# Autodesk Inventor assembly: Top_Slider Assy
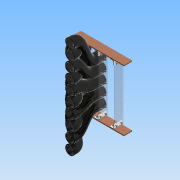
[picture p0: Inventor's stored thumbnail of the model, 180x180]
Saved by Autodesk Inventor 2018.1 (Build 221171000, 171)
## iProperties
Created: 2019-03-18
Part Number: Top_Slider Assy
Document SubType Name: Assembly
Designer: James
Author: James
## Documents named in this file (18)
- C:\Users\admin\Desktop\Ball-Machine\Top Level\Top_Slider Assy.iam
- C:\Users\admin\Desktop\Ball-Machine\Top Level\Top_Slider Piece 1.ipt
- C:\Users\admin\Desktop\Ball-Machine\Top Level\Top_Slider Piece 2.ipt
- C:\Users\admin\Desktop\Ball-Machine\Timing Gate\Timing_Angle Bracket.ipt
- C:\Users\admin\Desktop\Ball-Machine\Timing Gate\Nyloc Nut - M4.ipt
- C:\Users\admin\Desktop\Ball-Machine\Selection Sort\Socket Csk Screw - (A2) - M4 x  12.ipt
- C:\Users\admin\Desktop\Ball-Machine\Top Level\Pipes\Top_Pipe 01.ipt
- C:\Users\admin\Desktop\Ball-Machine\Top Level\Pipes\Top_Pipe 02.ipt
- C:\Users\admin\Desktop\Ball-Machine\Top Level\Pipes\Top_Pipe 03.ipt
- C:\Users\admin\Desktop\Ball-Machine\Top Level\Pipes\Top_Pipe 04.ipt
- C:\Users\admin\Desktop\Ball-Machine\Top Level\Pipes\Top_Pipe 05.ipt
- C:\Users\admin\Desktop\Ball-Machine\Top Level\Pipes\Top_Pipe 06.ipt
- C:\Users\admin\Desktop\Ball-Machine\Top Level\Pipes\Top_Pipe 07.ipt
- C:\Users\admin\Desktop\Ball-Machine\Top Level\Pipes\Top_Pipe 08.ipt
- C:\Users\admin\Desktop\Ball-Machine\Top Level\Pipes\Top_Pipe 09.ipt
- C:\Users\admin\Desktop\Ball-Machine\Top Level\Pipes\Top_Pipe 10.ipt
- C:\Users\admin\Desktop\Ball-Machine\Selection Sort\Socket Csk Screw - (A2) - M4 x  16.ipt
- C:\Users\admin\Desktop\Ball-Machine\Selection Sort\Socket Cap Screw - Standard - (A2) - M4 x 16.ipt
## Components (109 placed, 17 different names)
1. Top_Slider Piece 1:1 — Mate:1, Mate:2, Flush:6, Flush:7, Mate:25, Mate:75, Mate:76, Tangent:18, Angle:6, Mate:77, Mate:78, Tangent:19, Angle:7, Mate:79, Mate:80, Tangent:20, Angle:8, Mate:81, Mate:82, Tangent:21, Angle:9, Mate:83, Mate:84, Tangent:22, Angle:10, Mate:85, Mate:86, Flush:26, Mate:89, Mate:90, Mate:123, Mate:134
2. Top_Slider Piece 2:1 — Flush:1, Flush:2, Flush:3, Mate:1, Flush:4, Flush:5, Flush:6, Mate:3, Mate:4, Mate:11, Mate:12, Mate:13, Mate:14, Mate:15, Mate:16, Mate:17, Mate:18, Mate:19, Mate:60, Mate:61, Mate:62, Mate:63, Mate:64, Tangent:2, Tangent:3, Tangent:4, Tangent:5, Tangent:10, Tangent:12
3. Top_Slider Piece 1:2 — Flush:7, Flush:8, Mate:3, Mate:24, Mate:65, Mate:66, Tangent:13, Mate:67, Mate:68, Mate:69, Mate:70, Mate:71, Mate:72, Mate:73, Mate:74, Tangent:14, Tangent:15, Tangent:16, Tangent:17, Angle:2, Angle:3, Angle:4, Angle:5, Mate:87, Mate:88, Flush:24, Mate:91, Mate:92, Mate:124, Mate:125, Mate:129, Mate:132, Mate:135, Mate:138
4. Top_Slider Piece 1:3 — Flush:8, Mate:4, Mate:23, Mate:126, Mate:127, Mate:128, Mate:133, Mate:136, Mate:137
5. Top_Slider Piece 2:2 — Mate:2, Flush:4, Flush:5, Mate:5, Mate:6, Mate:7, Flush:9, Flush:10, Mate:8, Mate:9, Mate:10, Mate:20, Mate:21, Mate:22, Mate:27, Tangent:1, Tangent:6, Tangent:7, Tangent:8, Tangent:9, Tangent:11
6. Nyloc Nut - M4:34 — Mate:97, Mate:98
7. Socket Cap Screw - Standard - (A2) - M4 x 16:1 — Mate:97, Mate:98, Flush:27, Mate:121, Mate:123
8. Nyloc Nut - M4:35
9. Socket Cap Screw - Standard - (A2) - M4 x 16:2 — Flush:27, Mate:122
10. Nyloc Nut - M4:36
11. Socket Cap Screw - Standard - (A2) - M4 x 16:3 — Flush:28, Mate:124, Mate:138
12. Nyloc Nut - M4:37
13. Socket Cap Screw - Standard - (A2) - M4 x 16:4 — Flush:28, Mate:125
14. Nyloc Nut - M4:38
15. Socket Cap Screw - Standard - (A2) - M4 x 16:5 — Flush:29, Mate:126, Mate:137
16. Nyloc Nut - M4:39
17. Socket Cap Screw - Standard - (A2) - M4 x 16:6 — Flush:29, Mate:127
18. Nyloc Nut - M4:40
19. Socket Cap Screw - Standard - (A2) - M4 x 16:7 — Flush:30, Mate:129, Mate:135
20. Nyloc Nut - M4:41
21. Socket Cap Screw - Standard - (A2) - M4 x 16:8 — Flush:30, Mate:132
22. Nyloc Nut - M4:42
23. Socket Cap Screw - Standard - (A2) - M4 x 16:9 — Flush:31, Mate:130, Mate:134
24. Nyloc Nut - M4:43
25. Socket Cap Screw - Standard - (A2) - M4 x 16:10 — Flush:31, Mate:131
26. Nyloc Nut - M4:44
27. Socket Cap Screw - Standard - (A2) - M4 x 16:11 — Flush:32, Mate:128, Mate:136
28. Nyloc Nut - M4:45
29. Socket Cap Screw - Standard - (A2) - M4 x 16:12 — Flush:32, Mate:133
30. Timing_Angle Bracket:1 — Mate:5, Mate:6, Mate:7, Flush:9, Flush:10, Mate:25, Mate:29, Mate:54, Mate:121, Mate:122
31. Timing_Angle Bracket:2 — Mate:8, Mate:9, Mate:10, Mate:24, Mate:55, Mate:56
32. Timing_Angle Bracket:3 — Mate:11, Mate:12, Mate:13, Mate:59, Mate:130, Mate:131
33. Timing_Angle Bracket:4 — Mate:14, Mate:15, Mate:16
34. Timing_Angle Bracket:5 — Mate:20, Mate:21, Mate:22, Mate:23, Mate:57, Mate:58
35. Timing_Angle Bracket:6 — Mate:17, Mate:18, Mate:19
36. Nyloc Nut - M4:1 — Mate:28, Mate:29
37. Socket Csk Screw - (A2) - M4 x  12:1 — Mate:27, Tangent:1, Mate:28
38. Nyloc Nut - M4:2 — Flush:11, Mate:31
39. Socket Csk Screw - (A2) - M4 x  12:2 — Flush:11, Mate:31, Mate:54, Tangent:6
40. Nyloc Nut - M4:3
41. Socket Csk Screw - (A2) - M4 x  12:3 — Mate:55, Tangent:7
42. Nyloc Nut - M4:4
43. Socket Csk Screw - (A2) - M4 x  12:4 — Mate:56, Tangent:8
44. Nyloc Nut - M4:5
45. Socket Csk Screw - (A2) - M4 x  12:5 — Mate:57, Tangent:11
46. Nyloc Nut - M4:6
47. Socket Csk Screw - (A2) - M4 x  12:6 — Mate:64, Tangent:12
48. Nyloc Nut - M4:8
49. Socket Csk Screw - (A2) - M4 x  12:8 — Mate:58, Tangent:9
50. Nyloc Nut - M4:9
51. Socket Csk Screw - (A2) - M4 x  12:9 — Mate:63, Tangent:10
52. Nyloc Nut - M4:10
53. Socket Csk Screw - (A2) - M4 x  12:10 — Mate:61, Tangent:2
54. Nyloc Nut - M4:11
55. Socket Csk Screw - (A2) - M4 x  12:11 — Mate:62, Tangent:3
56. Nyloc Nut - M4:12
57. Socket Csk Screw - (A2) - M4 x  12:12 — Mate:60, Tangent:5
58. Nyloc Nut - M4:13
59. Socket Csk Screw - (A2) - M4 x  12:13 — Mate:59, Tangent:4
60. Top_Pipe 01:1 — Mate:65, Mate:66, Tangent:13, Angle:1
61. Top_Pipe 02:1 — Mate:67, Mate:68, Tangent:17, Angle:2
62. Top_Pipe 03:1 — Mate:69, Mate:70, Tangent:16, Angle:3
63. Top_Pipe 04:1 — Mate:71, Mate:72, Tangent:15, Angle:4
64. Top_Pipe 05:1 — Mate:73, Mate:74, Tangent:14, Angle:5
65. Top_Pipe 06:1 — Mate:75, Mate:76, Tangent:18, Angle:6
66. Top_Pipe 07:1 — Mate:77, Mate:78, Tangent:19, Angle:7
67. Top_Pipe 08:1 — Mate:79, Mate:80, Tangent:20, Angle:8
68. Top_Pipe 09:1 — Mate:81, Mate:82, Tangent:21, Angle:9
69. Top_Pipe 10:1 — Mate:83, Mate:84, Tangent:22, Angle:10
70. Socket Csk Screw - (A2) - M4 x  16:3 — Mate:87, Flush:23, Flush:24, Mate:93
71. Socket Csk Screw - (A2) - M4 x  16:4 — Mate:88, Flush:23, Mate:94
72. Nyloc Nut - M4:15 — Mate:89, Mate:95
73. Socket Csk Screw - (A2) - M4 x  16:1 — Mate:85, Flush:25, Flush:26, Mate:95
74. Nyloc Nut - M4:14 — Mate:90, Mate:96
75. Socket Csk Screw - (A2) - M4 x  16:2 — Mate:86, Flush:25, Mate:96
76. Nyloc Nut - M4:17 — Mate:92, Mate:94
77. Nyloc Nut - M4:16 — Mate:91, Mate:93
78. Socket Csk Screw - (A2) - M4 x  16:5
79. Socket Csk Screw - (A2) - M4 x  16:6
80. Nyloc Nut - M4:18
81. Socket Csk Screw - (A2) - M4 x  16:7
82. Nyloc Nut - M4:19
83. Socket Csk Screw - (A2) - M4 x  16:8
84. Nyloc Nut - M4:20
85. Nyloc Nut - M4:21
86. Socket Csk Screw - (A2) - M4 x  16:9
87. Socket Csk Screw - (A2) - M4 x  16:10
88. Nyloc Nut - M4:22
89. Socket Csk Screw - (A2) - M4 x  16:11
90. Nyloc Nut - M4:23
91. Socket Csk Screw - (A2) - M4 x  16:12
92. Nyloc Nut - M4:24
93. Nyloc Nut - M4:25
94. Socket Csk Screw - (A2) - M4 x  16:13
95. Socket Csk Screw - (A2) - M4 x  16:14
96. Nyloc Nut - M4:26
97. Socket Csk Screw - (A2) - M4 x  16:15
98. Nyloc Nut - M4:27
99. Socket Csk Screw - (A2) - M4 x  16:16
100. Nyloc Nut - M4:28
101. Nyloc Nut - M4:29
102. Socket Csk Screw - (A2) - M4 x  16:17
103. Socket Csk Screw - (A2) - M4 x  16:18
104. Nyloc Nut - M4:30
105. Socket Csk Screw - (A2) - M4 x  16:19
106. Nyloc Nut - M4:31
107. Socket Csk Screw - (A2) - M4 x  16:20
108. Nyloc Nut - M4:32
109. Nyloc Nut - M4:33
## Component patterns: (5 elements, first: Socket Csk Screw - (A2) - M4 x  16:3 + Socket Csk Screw - (A2) - M4 x  16:4 + Nyloc Nut - M4:15 + Socket Csk Screw - (A2) - M4 x  16:1 + Nyloc Nut - M4:14 + Socket Csk Screw - (A2) - M4 x  16:2 + Nyloc Nut - M4:17 + Nyloc Nut - M4:16)
## Relationships (198: Mate 135, Flush 31, Tangent 22, Angle 10)
- Flush:1: Top_Slider Piece 2:1
- Flush:2: Top_Slider Piece 2:1
- Flush:3: Top_Slider Piece 2:1
- Mate:1: Top_Slider Piece 1:1 ↔ Top_Slider Piece 2:1
- Mate:2: Top_Slider Piece 1:1 ↔ Top_Slider Piece 2:2
- Flush:4: Top_Slider Piece 2:1 ↔ Top_Slider Piece 2:2
- Flush:5: Top_Slider Piece 2:1 ↔ Top_Slider Piece 2:2
- Flush:6: Top_Slider Piece 1:1 ↔ Top_Slider Piece 2:1
- Flush:7: Top_Slider Piece 1:1 ↔ Top_Slider Piece 1:2
- Flush:8: Top_Slider Piece 1:2 ↔ Top_Slider Piece 1:3
- Mate:3: Top_Slider Piece 2:1 ↔ Top_Slider Piece 1:2
- Mate:4: Top_Slider Piece 2:1 ↔ Top_Slider Piece 1:3
- Mate:5: Top_Slider Piece 2:2 ↔ Timing_Angle Bracket:1
- Mate:6: Top_Slider Piece 2:2 ↔ Timing_Angle Bracket:1
- Mate:7: Top_Slider Piece 2:2 ↔ Timing_Angle Bracket:1
- Flush:9: Top_Slider Piece 2:2 ↔ Timing_Angle Bracket:1
- Flush:10: Top_Slider Piece 2:2 ↔ Timing_Angle Bracket:1
- Mate:8: Top_Slider Piece 2:2 ↔ Timing_Angle Bracket:2
- Mate:9: Top_Slider Piece 2:2 ↔ Timing_Angle Bracket:2
- Mate:10: Top_Slider Piece 2:2 ↔ Timing_Angle Bracket:2
- Mate:11: Top_Slider Piece 2:1 ↔ Timing_Angle Bracket:3
- Mate:12: Top_Slider Piece 2:1 ↔ Timing_Angle Bracket:3
- Mate:13: Top_Slider Piece 2:1 ↔ Timing_Angle Bracket:3
- Mate:14: Top_Slider Piece 2:1 ↔ Timing_Angle Bracket:4
- Mate:15: Top_Slider Piece 2:1 ↔ Timing_Angle Bracket:4
- Mate:16: Top_Slider Piece 2:1 ↔ Timing_Angle Bracket:4
- Mate:17: Top_Slider Piece 2:1 ↔ Timing_Angle Bracket:6
- Mate:18: Top_Slider Piece 2:1 ↔ Timing_Angle Bracket:6
- Mate:19: Top_Slider Piece 2:1 ↔ Timing_Angle Bracket:6
- Mate:20: Top_Slider Piece 2:2 ↔ Timing_Angle Bracket:5
- Mate:21: Top_Slider Piece 2:2 ↔ Timing_Angle Bracket:5
- Mate:22: Top_Slider Piece 2:2 ↔ Timing_Angle Bracket:5
- Mate:23: Top_Slider Piece 1:3 ↔ Timing_Angle Bracket:5
- Mate:24: Top_Slider Piece 1:2 ↔ Timing_Angle Bracket:2
- Mate:25: Top_Slider Piece 1:1 ↔ Timing_Angle Bracket:1
- Mate:27: Top_Slider Piece 2:2 ↔ Socket Csk Screw - (A2) - M4 x  12:1
- Tangent:1: Top_Slider Piece 2:2 ↔ Socket Csk Screw - (A2) - M4 x  12:1
- Mate:28: Nyloc Nut - M4:1 ↔ Socket Csk Screw - (A2) - M4 x  12:1
- Mate:29: Timing_Angle Bracket:1 ↔ Nyloc Nut - M4:1
- [Mate]: Nyloc Nut - M4:2 ↔ Socket Csk Screw - (A2) - M4 x  12:2
- Flush:11 (7.78 mm): Nyloc Nut - M4:2 ↔ Socket Csk Screw - (A2) - M4 x  12:2
- Mate:31: Nyloc Nut - M4:2 ↔ Socket Csk Screw - (A2) - M4 x  12:2
- [Mate]: Nyloc Nut - M4:3 ↔ Socket Csk Screw - (A2) - M4 x  12:3
- [Flush] (7.78 mm): Nyloc Nut - M4:3 ↔ Socket Csk Screw - (A2) - M4 x  12:3
- [Mate]: Nyloc Nut - M4:3 ↔ Socket Csk Screw - (A2) - M4 x  12:3
- [Mate]: Nyloc Nut - M4:4 ↔ Socket Csk Screw - (A2) - M4 x  12:4
- [Flush] (7.78 mm): Nyloc Nut - M4:4 ↔ Socket Csk Screw - (A2) - M4 x  12:4
- [Mate]: Nyloc Nut - M4:4 ↔ Socket Csk Screw - (A2) - M4 x  12:4
- [Mate]: Nyloc Nut - M4:5 ↔ Socket Csk Screw - (A2) - M4 x  12:5
- [Flush] (7.78 mm): Nyloc Nut - M4:5 ↔ Socket Csk Screw - (A2) - M4 x  12:5
- [Mate]: Nyloc Nut - M4:5 ↔ Socket Csk Screw - (A2) - M4 x  12:5
- [Mate]: Nyloc Nut - M4:6 ↔ Socket Csk Screw - (A2) - M4 x  12:6
- [Flush] (7.78 mm): Nyloc Nut - M4:6 ↔ Socket Csk Screw - (A2) - M4 x  12:6
- [Mate]: Nyloc Nut - M4:6 ↔ Socket Csk Screw - (A2) - M4 x  12:6
- [Mate]: Nyloc Nut - M4:8 ↔ Socket Csk Screw - (A2) - M4 x  12:8
- [Flush] (7.78 mm): Nyloc Nut - M4:8 ↔ Socket Csk Screw - (A2) - M4 x  12:8
- [Mate]: Nyloc Nut - M4:8 ↔ Socket Csk Screw - (A2) - M4 x  12:8
- [Mate]: Nyloc Nut - M4:9 ↔ Socket Csk Screw - (A2) - M4 x  12:9
- [Flush] (7.78 mm): Nyloc Nut - M4:9 ↔ Socket Csk Screw - (A2) - M4 x  12:9
- [Mate]: Nyloc Nut - M4:9 ↔ Socket Csk Screw - (A2) - M4 x  12:9
- [Mate]: Nyloc Nut - M4:10 ↔ Socket Csk Screw - (A2) - M4 x  12:10
- [Flush] (7.78 mm): Nyloc Nut - M4:10 ↔ Socket Csk Screw - (A2) - M4 x  12:10
- [Mate]: Nyloc Nut - M4:10 ↔ Socket Csk Screw - (A2) - M4 x  12:10
- [Mate]: Nyloc Nut - M4:11 ↔ Socket Csk Screw - (A2) - M4 x  12:11
- [Flush] (7.78 mm): Nyloc Nut - M4:11 ↔ Socket Csk Screw - (A2) - M4 x  12:11
- [Mate]: Nyloc Nut - M4:11 ↔ Socket Csk Screw - (A2) - M4 x  12:11
- [Mate]: Nyloc Nut - M4:12 ↔ Socket Csk Screw - (A2) - M4 x  12:12
- [Flush] (7.78 mm): Nyloc Nut - M4:12 ↔ Socket Csk Screw - (A2) - M4 x  12:12
- [Mate]: Nyloc Nut - M4:12 ↔ Socket Csk Screw - (A2) - M4 x  12:12
- [Mate]: Nyloc Nut - M4:13 ↔ Socket Csk Screw - (A2) - M4 x  12:13
- [Flush] (7.78 mm): Nyloc Nut - M4:13 ↔ Socket Csk Screw - (A2) - M4 x  12:13
- [Mate]: Nyloc Nut - M4:13 ↔ Socket Csk Screw - (A2) - M4 x  12:13
- Mate:54: Timing_Angle Bracket:1 ↔ Socket Csk Screw - (A2) - M4 x  12:2
- Mate:55: Timing_Angle Bracket:2 ↔ Socket Csk Screw - (A2) - M4 x  12:3
- Mate:56: Timing_Angle Bracket:2 ↔ Socket Csk Screw - (A2) - M4 x  12:4
- Mate:57: Timing_Angle Bracket:5 ↔ Socket Csk Screw - (A2) - M4 x  12:5
- Mate:58: Timing_Angle Bracket:5 ↔ Socket Csk Screw - (A2) - M4 x  12:8
- Mate:59: Timing_Angle Bracket:3 ↔ Socket Csk Screw - (A2) - M4 x  12:13
- Mate:60: Top_Slider Piece 2:1 ↔ Socket Csk Screw - (A2) - M4 x  12:12
- Mate:61: Top_Slider Piece 2:1 ↔ Socket Csk Screw - (A2) - M4 x  12:10
- Mate:62: Top_Slider Piece 2:1 ↔ Socket Csk Screw - (A2) - M4 x  12:11
- Mate:63: Top_Slider Piece 2:1 ↔ Socket Csk Screw - (A2) - M4 x  12:9
- Mate:64: Top_Slider Piece 2:1 ↔ Socket Csk Screw - (A2) - M4 x  12:6
- Tangent:2: Top_Slider Piece 2:1 ↔ Socket Csk Screw - (A2) - M4 x  12:10
- Tangent:3: Top_Slider Piece 2:1 ↔ Socket Csk Screw - (A2) - M4 x  12:11
- Tangent:4: Top_Slider Piece 2:1 ↔ Socket Csk Screw - (A2) - M4 x  12:13
- Tangent:5: Top_Slider Piece 2:1 ↔ Socket Csk Screw - (A2) - M4 x  12:12
- Tangent:6: Top_Slider Piece 2:2 ↔ Socket Csk Screw - (A2) - M4 x  12:2
- Tangent:7: Top_Slider Piece 2:2 ↔ Socket Csk Screw - (A2) - M4 x  12:3
- Tangent:8: Top_Slider Piece 2:2 ↔ Socket Csk Screw - (A2) - M4 x  12:4
- Tangent:9: Top_Slider Piece 2:2 ↔ Socket Csk Screw - (A2) - M4 x  12:8
- Tangent:10: Top_Slider Piece 2:1 ↔ Socket Csk Screw - (A2) - M4 x  12:9
- Tangent:11: Top_Slider Piece 2:2 ↔ Socket Csk Screw - (A2) - M4 x  12:5
- Tangent:12: Top_Slider Piece 2:1 ↔ Socket Csk Screw - (A2) - M4 x  12:6
- Mate:65: Top_Slider Piece 1:2 ↔ Top_Pipe 01:1
- Mate:66: Top_Slider Piece 1:2 ↔ Top_Pipe 01:1
- Tangent:13: Top_Slider Piece 1:2 ↔ Top_Pipe 01:1
- Angle:1 (180 deg): Top_Pipe 01:1
- Mate:67: Top_Slider Piece 1:2 ↔ Top_Pipe 02:1
- Mate:68: Top_Slider Piece 1:2 ↔ Top_Pipe 02:1
- Mate:69: Top_Slider Piece 1:2 ↔ Top_Pipe 03:1
- Mate:70: Top_Slider Piece 1:2 ↔ Top_Pipe 03:1
- Mate:71: Top_Slider Piece 1:2 ↔ Top_Pipe 04:1
- Mate:72: Top_Slider Piece 1:2 ↔ Top_Pipe 04:1
- Mate:73: Top_Slider Piece 1:2 ↔ Top_Pipe 05:1
- Mate:74: Top_Slider Piece 1:2 ↔ Top_Pipe 05:1
- Tangent:14: Top_Slider Piece 1:2 ↔ Top_Pipe 05:1
- Tangent:15: Top_Slider Piece 1:2 ↔ Top_Pipe 04:1
- Tangent:16: Top_Slider Piece 1:2 ↔ Top_Pipe 03:1
- Tangent:17: Top_Slider Piece 1:2 ↔ Top_Pipe 02:1
- Angle:2 (0 deg): Top_Slider Piece 1:2 ↔ Top_Pipe 02:1
- Angle:3 (0 deg): Top_Slider Piece 1:2 ↔ Top_Pipe 03:1
- Angle:4 (0 deg): Top_Slider Piece 1:2 ↔ Top_Pipe 04:1
- Angle:5 (0 deg): Top_Slider Piece 1:2 ↔ Top_Pipe 05:1
- Mate:75: Top_Slider Piece 1:1 ↔ Top_Pipe 06:1
- Mate:76: Top_Slider Piece 1:1 ↔ Top_Pipe 06:1
- Tangent:18: Top_Slider Piece 1:1 ↔ Top_Pipe 06:1
- Angle:6 (180 deg): Top_Slider Piece 1:1 ↔ Top_Pipe 06:1
- Mate:77: Top_Slider Piece 1:1 ↔ Top_Pipe 07:1
- Mate:78: Top_Slider Piece 1:1 ↔ Top_Pipe 07:1
- Tangent:19: Top_Slider Piece 1:1 ↔ Top_Pipe 07:1
- Angle:7 (0 deg): Top_Slider Piece 1:1 ↔ Top_Pipe 07:1
- Mate:79: Top_Slider Piece 1:1 ↔ Top_Pipe 08:1
- Mate:80: Top_Slider Piece 1:1 ↔ Top_Pipe 08:1
- Tangent:20: Top_Slider Piece 1:1 ↔ Top_Pipe 08:1
- Angle:8 (0 deg): Top_Slider Piece 1:1 ↔ Top_Pipe 08:1
- Mate:81: Top_Slider Piece 1:1 ↔ Top_Pipe 09:1
- Mate:82: Top_Slider Piece 1:1 ↔ Top_Pipe 09:1
- Tangent:21: Top_Slider Piece 1:1 ↔ Top_Pipe 09:1
- Angle:9 (0 deg): Top_Slider Piece 1:1 ↔ Top_Pipe 09:1
- Mate:83: Top_Slider Piece 1:1 ↔ Top_Pipe 10:1
- Mate:84: Top_Slider Piece 1:1 ↔ Top_Pipe 10:1
- Tangent:22: Top_Slider Piece 1:1 ↔ Top_Pipe 10:1
- Angle:10 (0 deg): Top_Slider Piece 1:1 ↔ Top_Pipe 10:1
- Mate:85: Top_Slider Piece 1:1 ↔ Socket Csk Screw - (A2) - M4 x  16:1
- Mate:86: Top_Slider Piece 1:1 ↔ Socket Csk Screw - (A2) - M4 x  16:2
- Mate:87: Top_Slider Piece 1:2 ↔ Socket Csk Screw - (A2) - M4 x  16:3
- Mate:88: Top_Slider Piece 1:2 ↔ Socket Csk Screw - (A2) - M4 x  16:4
- Flush:23: Socket Csk Screw - (A2) - M4 x  16:3 ↔ Socket Csk Screw - (A2) - M4 x  16:4
- Flush:24 (-5 mm): Top_Slider Piece 1:2 ↔ Socket Csk Screw - (A2) - M4 x  16:3
- Flush:25: Socket Csk Screw - (A2) - M4 x  16:1 ↔ Socket Csk Screw - (A2) - M4 x  16:2
- Flush:26 (-5 mm): Top_Slider Piece 1:1 ↔ Socket Csk Screw - (A2) - M4 x  16:1
- Mate:89: Top_Slider Piece 1:1 ↔ Nyloc Nut - M4:15
- Mate:90: Top_Slider Piece 1:1 ↔ Nyloc Nut - M4:14
- Mate:91: Top_Slider Piece 1:2 ↔ Nyloc Nut - M4:16
- Mate:92: Top_Slider Piece 1:2 ↔ Nyloc Nut - M4:17
- Mate:93: Socket Csk Screw - (A2) - M4 x  16:3 ↔ Nyloc Nut - M4:16
- Mate:94: Socket Csk Screw - (A2) - M4 x  16:4 ↔ Nyloc Nut - M4:17
- Mate:95: Nyloc Nut - M4:15 ↔ Socket Csk Screw - (A2) - M4 x  16:1
- Mate:96: Nyloc Nut - M4:14 ↔ Socket Csk Screw - (A2) - M4 x  16:2
- Mate:97: Nyloc Nut - M4:34 ↔ Socket Cap Screw - Standard - (A2) - M4 x 16:1
- Mate:98 (8 mm): Nyloc Nut - M4:34 ↔ Socket Cap Screw - Standard - (A2) - M4 x 16:1
- [Mate]: Nyloc Nut - M4:35 ↔ Socket Cap Screw - Standard - (A2) - M4 x 16:2
- [Mate] (8 mm): Nyloc Nut - M4:35 ↔ Socket Cap Screw - Standard - (A2) - M4 x 16:2
- [Mate]: Nyloc Nut - M4:36 ↔ Socket Cap Screw - Standard - (A2) - M4 x 16:3
- [Mate] (8 mm): Nyloc Nut - M4:36 ↔ Socket Cap Screw - Standard - (A2) - M4 x 16:3
- [Mate]: Nyloc Nut - M4:37 ↔ Socket Cap Screw - Standard - (A2) - M4 x 16:4
- [Mate] (8 mm): Nyloc Nut - M4:37 ↔ Socket Cap Screw - Standard - (A2) - M4 x 16:4
- [Mate]: Nyloc Nut - M4:38 ↔ Socket Cap Screw - Standard - (A2) - M4 x 16:5
- [Mate] (8 mm): Nyloc Nut - M4:38 ↔ Socket Cap Screw - Standard - (A2) - M4 x 16:5
- [Mate]: Nyloc Nut - M4:39 ↔ Socket Cap Screw - Standard - (A2) - M4 x 16:6
- [Mate] (8 mm): Nyloc Nut - M4:39 ↔ Socket Cap Screw - Standard - (A2) - M4 x 16:6
- [Mate]: Nyloc Nut - M4:40 ↔ Socket Cap Screw - Standard - (A2) - M4 x 16:7
- [Mate] (8 mm): Nyloc Nut - M4:40 ↔ Socket Cap Screw - Standard - (A2) - M4 x 16:7
- [Mate]: Nyloc Nut - M4:41 ↔ Socket Cap Screw - Standard - (A2) - M4 x 16:8
- [Mate] (8 mm): Nyloc Nut - M4:41 ↔ Socket Cap Screw - Standard - (A2) - M4 x 16:8
- [Mate]: Nyloc Nut - M4:42 ↔ Socket Cap Screw - Standard - (A2) - M4 x 16:9
- [Mate] (8 mm): Nyloc Nut - M4:42 ↔ Socket Cap Screw - Standard - (A2) - M4 x 16:9
- [Mate]: Nyloc Nut - M4:43 ↔ Socket Cap Screw - Standard - (A2) - M4 x 16:10
- [Mate] (8 mm): Nyloc Nut - M4:43 ↔ Socket Cap Screw - Standard - (A2) - M4 x 16:10
- [Mate]: Nyloc Nut - M4:44 ↔ Socket Cap Screw - Standard - (A2) - M4 x 16:11
- [Mate] (8 mm): Nyloc Nut - M4:44 ↔ Socket Cap Screw - Standard - (A2) - M4 x 16:11
- [Mate]: Nyloc Nut - M4:45 ↔ Socket Cap Screw - Standard - (A2) - M4 x 16:12
- [Mate] (8 mm): Nyloc Nut - M4:45 ↔ Socket Cap Screw - Standard - (A2) - M4 x 16:12
- Flush:27: Socket Cap Screw - Standard - (A2) - M4 x 16:1 ↔ Socket Cap Screw - Standard - (A2) - M4 x 16:2
- Mate:121: Socket Cap Screw - Standard - (A2) - M4 x 16:1 ↔ Timing_Angle Bracket:1
- Mate:122: Socket Cap Screw - Standard - (A2) - M4 x 16:2 ↔ Timing_Angle Bracket:1
- Mate:123: Top_Slider Piece 1:1 ↔ Socket Cap Screw - Standard - (A2) - M4 x 16:1
- Flush:28: Socket Cap Screw - Standard - (A2) - M4 x 16:3 ↔ Socket Cap Screw - Standard - (A2) - M4 x 16:4
- Flush:29: Socket Cap Screw - Standard - (A2) - M4 x 16:5 ↔ Socket Cap Screw - Standard - (A2) - M4 x 16:6
- Mate:124: Top_Slider Piece 1:2 ↔ Socket Cap Screw - Standard - (A2) - M4 x 16:3
- Mate:125: Top_Slider Piece 1:2 ↔ Socket Cap Screw - Standard - (A2) - M4 x 16:4
- Mate:126: Top_Slider Piece 1:3 ↔ Socket Cap Screw - Standard - (A2) - M4 x 16:5
- Mate:127: Top_Slider Piece 1:3 ↔ Socket Cap Screw - Standard - (A2) - M4 x 16:6
- Flush:30: Socket Cap Screw - Standard - (A2) - M4 x 16:7 ↔ Socket Cap Screw - Standard - (A2) - M4 x 16:8
- Flush:31: Socket Cap Screw - Standard - (A2) - M4 x 16:9 ↔ Socket Cap Screw - Standard - (A2) - M4 x 16:10
- Flush:32: Socket Cap Screw - Standard - (A2) - M4 x 16:11 ↔ Socket Cap Screw - Standard - (A2) - M4 x 16:12
- Mate:128: Top_Slider Piece 1:3 ↔ Socket Cap Screw - Standard - (A2) - M4 x 16:11
- Mate:129: Top_Slider Piece 1:2 ↔ Socket Cap Screw - Standard - (A2) - M4 x 16:7
- Mate:130: Socket Cap Screw - Standard - (A2) - M4 x 16:9 ↔ Timing_Angle Bracket:3
- Mate:131: Socket Cap Screw - Standard - (A2) - M4 x 16:10 ↔ Timing_Angle Bracket:3
- Mate:132: Top_Slider Piece 1:2 ↔ Socket Cap Screw - Standard - (A2) - M4 x 16:8
- Mate:133: Top_Slider Piece 1:3 ↔ Socket Cap Screw - Standard - (A2) - M4 x 16:12
- Mate:134: Top_Slider Piece 1:1 ↔ Socket Cap Screw - Standard - (A2) - M4 x 16:9
- Mate:135: Top_Slider Piece 1:2 ↔ Socket Cap Screw - Standard - (A2) - M4 x 16:7
- Mate:136: Top_Slider Piece 1:3 ↔ Socket Cap Screw - Standard - (A2) - M4 x 16:11
- Mate:137: Top_Slider Piece 1:3 ↔ Socket Cap Screw - Standard - (A2) - M4 x 16:5
- Mate:138: Top_Slider Piece 1:2 ↔ Socket Cap Screw - Standard - (A2) - M4 x 16:3
## Named parameters: d41_d39 = 0 mm, d44_d41_d39 = 0 mm, d45_d42 = 7.78 mm, d46_d43 = 0 mm, d47_d41_d39 = 0 mm, d48_d42 = 7.78 mm, d49_d43 = 0 mm, d50_d41_d39 = 0 mm, d51_d42 = 7.78 mm, d52_d43 = 0 mm, d53_d41_d39 = 0 mm, d54_d42 = 7.78 mm, d55_d43 = 0 mm, d59_d41_d39 = 0 mm, d60_d42 = 7.78 mm, d61_d43 = 0 mm, d62_d41_d39 = 0 mm, d63_d42 = 7.78 mm, d64_d43 = 0 mm, d65_d41_d39 = 0 mm, d66_d42 = 7.78 mm, d67_d43 = 0 mm, d68_d41_d39 = 0 mm, d69_d42 = 7.78 mm, d70_d43 = 0 mm, d71_d41_d39 = 0 mm, d72_d42 = 7.78 mm, d73_d43 = 0 mm, d74_d41_d39 = 0 mm, d75_d42 = 7.78 mm, d76_d43 = 0 mm, d161_d159 = 0 mm, d162_d160 = 8 mm, d163_d159 = 0 mm, d164_d160 = 8 mm, d165_d159 = 0 mm, d166_d160 = 8 mm, d167_d159 = 0 mm, d168_d160 = 8 mm, d169_d159 = 0 mm, d170_d160 = 8 mm, d171_d159 = 0 mm, d172_d160 = 8 mm, d173_d159 = 0 mm, d174_d160 = 8 mm, d175_d159 = 0 mm, d176_d160 = 8 mm, d177_d159 = 0 mm, d178_d160 = 8 mm, d179_d159 = 0 mm, d180_d160 = 8 mm, d181_d159 = 0 mm, d182_d160 = 8 mm
